# Autodesk Inventor assembly: Assembly1
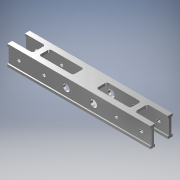
[picture p0: Inventor's stored thumbnail of the model, 180x180]
Saved by Autodesk Inventor 2017 (Build 210142000, 142)
## iProperties
Created: 2016-10-02
Part Number: Assembly1
Document SubType Name: Assembly
Designer: vslabsal
Author: vslabsal
## Documents named in this file (3)
- C:\Users\vslabsal\Documents\Assembly1.iam
- C:\Users\vslabsal\Documents\side cutout.ipt
- C:\Users\vslabsal\Documents\top cutout.ipt
## Components (4 placed, 2 different names)
1. side cutout:1 — Rigid:1
2. top cutout:1 — Rigid:1, Rigid:2
3. side cutout:2 — Rigid:2, Rigid:3
4. top cutout:2 — Rigid:3
## Relationships (3: WeldJoint 3)
- Rigid:1 [WeldJoint]: side cutout:1 ↔ top cutout:1
- Rigid:2 [WeldJoint]: top cutout:1 ↔ side cutout:2
- Rigid:3 [WeldJoint]: side cutout:2 ↔ top cutout:2
